# Autodesk Inventor assembly: 1808236 DFPI-100-280-ND2P-E-P-G2---(0)
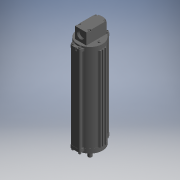
[picture p0: Inventor's stored thumbnail of the model, 180x180]
Saved by Autodesk Inventor 2017.3 (Build 213256000, 256)
## iProperties
Category: PARTsolutions
Company: FESTO
Part Number: 1808236 DFPI-100-280-ND2P-E-P-G2---(0)
Catalog Web Link: www.cadenas.de
Description: DFPI-Linear drive
Vendor: FESTO
Document SubType Name: Assembly
Designer: partserver
Manufacturer: FESTO
Mass: 5716 g
Surface Area: 3893.31 cm^2
Volume: 2228.04 cm^3
Density: 2.56549 g/cm^3
Title: 1808236 DFPI-100-280-ND2P-E-P-G2
Author: Cadenas PARTsolutions
Comments: Linear drive
PSOL_IDENT_0: {ATYP=ASSISTANT},{DATA=script=$CADENAS_DATA/23d-libs/festo/webfesto.vbb/&M_FAMILY=DFPI&M_GROUP=01&M_
PSOL_IDENT_1: PARTNO=1808236&IDCODE1=DFPI-100-280-ND2P-E-P-G2&IDCODE2=&HUB=280&customer_number_cns=&MATES=1&LOD=HI
PSOL_IDENT_2: &LOCKERP=0&SINGLEPART=1}
NB: 1808236 DFPI-100-280-ND2P-E-P-G2---(0)
NN: DFPI
NT: Linear drive
NBSYN: $TNR. $TYP.-$KDM.-$HUB.-$DF.$WS.$MF.$REGS.$AR1.$WV1.$NORM1.$ANS1.$SS1.$RM1.$GEN1.---($HUBST.)
LINA: 1808236 DFPI-100-280-ND2P-E-P-G2
CATALOG: Festo
OFFICIAL_STANDARD_NUMBERS: DIN 3358
TNR: 1808236
TYP: DFPI
KDM: 100
HUB: 280
HUBST: 0
DF: N
WS: D2
MF: P
REG: -
AR: E
WV: -
NORM: -
ANS: P
SS: -
RM: -
GEN: G2
AM: 32
B: 0
BA: 0
BG: 0
D1: 108
D2: 25
D3: 70
D4: 0
D5: M8
D6: -
D7: 0
D8: 119
E: 131
E1: 0
E2: 0
EA: 0
EB: 0
G: 0
J: 0
H1: 0
H2: 109
KK: M16x1.5
L0: 118.5
L1: 0
L2: 0
L5: 15
L6: 0
L8: 48.8
L9: 0.7
MM: 0
PL: 0
RT: -
SW: 0
SW1: 22
SW2: 0
TG: 0
VD: 0
VA: 0
WH: 16
ZB: 134.5
CNSMASSEXACT: 5.716
SUPPLIER: FESTO
ARTICLENO: 1808236 DFPI-100-280-ND2P-E-P-G2---(0)
BOMINFO: 1808236 DFPI-100-280-ND2P-E-P-G2
CREATOR: CADENAS GmbH
## Documents named in this file (3)
- e:\temp\worker_6\temp\exporttempdir_4476_176_D6oTJ\format_0\1808236 DFPI-100-280-ND2P-E-P-G2---(0).iam
- e:\temp\worker_6\temp\exporttempdir_4476_176_D6oTJ\format_0\1808236 DFPI-100-280-ND2P-E-P-G2(ZYL).ipt
- e:\temp\worker_6\temp\exporttempdir_4476_176_D6oTJ\format_0\1808236 DFPI-100-280-ND2P-E-P(K).ipt
## Components (2 placed, 2 different names)
1. 1808236 DFPI-100-280-ND2P-E-P-G2(ZYL):1 — TO_KOLBEN_Z@1 <-> KOLBEN_Z@2, TO_KOLBEN_YZ@1 <-> KOLBEN_YZ@2
2. 1808236 DFPI-100-280-ND2P-E-P(K):1 — TO_KOLBEN_Z@1 <-> KOLBEN_Z@2, TO_KOLBEN_YZ@1 <-> KOLBEN_YZ@2
## Relationships (2: Mate 1, Angle 1)
- TO_KOLBEN_Z@1 <-> KOLBEN_Z@2 [Mate]: 1808236 DFPI-100-280-ND2P-E-P-G2(ZYL):1 ↔ 1808236 DFPI-100-280-ND2P-E-P(K):1
- TO_KOLBEN_YZ@1 <-> KOLBEN_YZ@2 [Angle] (0 deg): 1808236 DFPI-100-280-ND2P-E-P-G2(ZYL):1 ↔ 1808236 DFPI-100-280-ND2P-E-P(K):1
